# Autodesk Inventor assembly: PhoneMountPivotAssembly
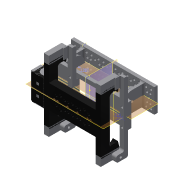
[picture p0: Inventor's stored thumbnail of the model, 180x180]
Saved by Autodesk Inventor 2018 (Build 220112000, 112)
## iProperties
Created: 2019-02-13
Part Number: PhoneMountPivotAssembly
Document SubType Name: Assembly
Designer: ball
Author: ball
## Documents named in this file (5)
- C:\FTC\FTC8863CAD\2018Robot\PhoneMountPivotAssembly.iam
- C:\FTC\FTC8863CAD\2018Robot\phone mount base.ipt
- C:\FTC\FTC8863CAD\2018Robot\phone mount pivot.ipt
- C:\FTC\FTC8863CAD\2018Robot\e4-phone_1piece pivot.ipt
- C:\FTC\FTC8863CAD\2018Robot\PhoneMountRightRib.ipt
## Components (5 placed, 4 different names)
1. phone mount base:1 — Mate:1, Mate:2
2. phone mount pivot:1 — Mate:1, Mate:2, Flush:1, Flush:2, Flush:3, Mate:5, Mate:6
3. e4-phone_1piece pivot:1 — Flush:1, Flush:2, Flush:3, Mate:3, Mate:4, Mate:7, Mate:8
4. PhoneMountRightRib:1 — Mate:3, Mate:4, Mate:5
5. PhoneMountRightRib:2 — Mate:6, Mate:7, Mate:8
## Relationships (11: Mate 8, Flush 3)
- Mate:1: phone mount base:1 ↔ phone mount pivot:1
- Mate:2 (0.254 mm): phone mount base:1 ↔ phone mount pivot:1
- Flush:1 (12.7 mm): phone mount pivot:1 ↔ e4-phone_1piece pivot:1
- Flush:2: phone mount pivot:1 ↔ e4-phone_1piece pivot:1
- Flush:3 (6.35 mm): phone mount pivot:1 ↔ e4-phone_1piece pivot:1
- Mate:3 (0.254 mm): e4-phone_1piece pivot:1 ↔ PhoneMountRightRib:1
- Mate:4: e4-phone_1piece pivot:1 ↔ PhoneMountRightRib:1
- Mate:5: phone mount pivot:1 ↔ PhoneMountRightRib:1
- Mate:6: phone mount pivot:1 ↔ PhoneMountRightRib:2
- Mate:7 (0.254 mm): e4-phone_1piece pivot:1 ↔ PhoneMountRightRib:2
- Mate:8: e4-phone_1piece pivot:1 ↔ PhoneMountRightRib:2
